# Autodesk Inventor assembly: Half Motor Sprocket Right
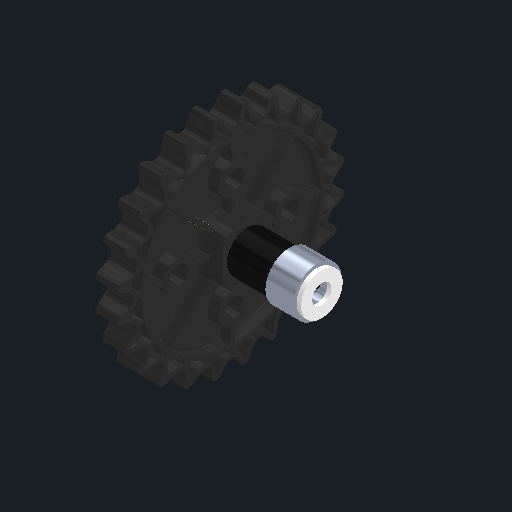
[picture p0: Inventor's stored thumbnail of the model, 512x512]
Saved by Autodesk Inventor 2025 (Build 290162000, 162)
## iProperties
Created: 2024-10-20
Part Number: Half Motor Sprocket Right
Document SubType Name: Assembly
Designer: Averey Ku
Author: Averey Ku
## Documents named in this file (9)
- D:\VEX\High Stakes\CAD\V2\Chassis\Drivebay Right\Half Motor Sprocket Right.iam
- D:\VEX\High Stakes\CAD\V2\Chassis\Drivebay Right\Shaft Collar Set Screw Right.ipt
- D:\vex_robotics_high_stakes\hardware\cad\robpros_cad_lib\Motion\Spacers\Washer Teflon\TWasher .375 OD x .04000.ipt
- D:\vex_robotics_high_stakes\hardware\cad\robpros_cad_lib\Motion\Spacers\Washer Teflon.ipt
- D:\vex_robotics_high_stakes\hardware\cad\robpros_cad_lib\Motion\Spacers\Washer Steel\SWasher .375 OD x .015625.ipt
- D:\vex_robotics_high_stakes\hardware\cad\robpros_cad_lib\Motion\Spacers\Washer Steel.ipt
- D:\VEX\High Stakes\CAD\V2\Chassis\Drivebay Right\6P 24T Sprocket, No Insert Right.iam
- D:\VEX\High Stakes\CAD\ROBOPROS-CAD-Inventor\Motion\Spacers\Spacer Nylon .375 OD\NSpacer .375 OD x .375.ipt
- D:\VEX\High Stakes\CAD\ROBOPROS-CAD-Inventor\Motion\Spacers\Spacer Nylon .375 OD.ipt
## Components (5 placed, 5 different names)
1. Shaft Collar Set Screw Right:1 — Insert:1, Insert:2, Insert:4
2. TWasher .375 OD x .04000:1 — Mate:1, Insert:1
3. SWasher .375 OD x .015625:1 — Insert:3
4. 6P 24T Sprocket, No Insert Right:1 [sub-assembly] — Insert:2, Insert:3
5. NSpacer .375 OD x .375:1 — Insert:4
## Relationships (5: Insert 4, Mate 1)
- Mate:1: TWasher .375 OD x .04000:1
- Insert:1: Shaft Collar Set Screw Right:1 ↔ TWasher .375 OD x .04000:1
- Insert:2 (9.525 mm): Shaft Collar Set Screw Right:1 ↔ 6P 24T Sprocket, No Insert Right:1
- Insert:3: SWasher .375 OD x .015625:1 ↔ 6P 24T Sprocket, No Insert Right:1
- Insert:4: Shaft Collar Set Screw Right:1 ↔ NSpacer .375 OD x .375:1
